# Autodesk Inventor assembly: BobbinGuide
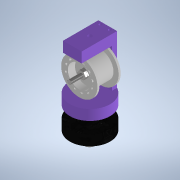
[picture p0: Inventor's stored thumbnail of the model, 180x180]
Saved by Autodesk Inventor 2020.2 (Build 242310000, 310)
## iProperties
Created: 2020-03-09
Part Number: BobbinGuide
Document SubType Name: Assembly
Designer: elmar
Author: elmar
## Documents named in this file (10)
- C:\Users\elmar\OneDrive\Inventor\FourWireBraidingMachine\Carriage.iam
- C:\Users\elmar\OneDrive\Inventor\FourWireBraidingMachine\CarriagePlate.ipt
- C:\Users\elmar\OneDrive\Inventor\FourWireBraidingMachine\SpoolHolder.ipt
- C:\Users\elmar\OneDrive\Inventor\FourWireBraidingMachine\Spool.ipt
- C:\Users\elmar\OneDrive\Inventor\FourWireBraidingMachine\Spring.ipt
- C:\Users\elmar\OneDrive\Documents\Inventor\Content Center Files\R2020\en-US\BS EN 24035\ISO 4035 - M3BS EN.ipt
- C:\Users\elmar\OneDrive\Documents\Inventor\Content Center Files\R2020\en-US\U 2494(1)\Unbrako - M3 x  30(6).ipt
- C:\Users\elmar\OneDrive\Inventor\FourWireBraidingMachine\CarriageGuide.ipt
- C:\Users\elmar\OneDrive\Inventor\FourWireBraidingMachine\SpoolSpringBushing.ipt
- C:\Users\elmar\OneDrive\Inventor\FourWireBraidingMachine\M8_34mmRod.ipt
## Components (10 placed, 9 different names)
1. CarriagePlate:1 — Insert:17
2. CarriageGuide:1
3. SpoolHolder:1 — Insert:14, Insert:15, Insert:16, Insert:17
4. Spool:1 — Mate:1, Mate:5, Insert:15
5. Spring:1 — Mate:1, Mate:5, Mate:6
6. SpoolSpringBushing:1 — Mate:6, Mate:7, Insert:13
7. BS EN 24035 - Metric M3:1 — Insert:9
8. BS EN 24035 - Metric M3:2 — Insert:9, Insert:13
9. Unbrako Hex Socket Cap - Metric M3 x 30:1 — Mate:7, Insert:14
10. M8_34mmRod:1 — Insert:16
## Relationships (10: Insert 6, Mate 4)
- Mate:1: Spool:1 ↔ Spring:1
- Insert:9: BS EN 24035 - Metric M3:1 ↔ BS EN 24035 - Metric M3:2
- Mate:5: Spool:1 ↔ Spring:1
- Mate:6: Spring:1 ↔ SpoolSpringBushing:1
- Mate:7: SpoolSpringBushing:1 ↔ Unbrako Hex Socket Cap - Metric M3 x 30:1
- Insert:13: SpoolSpringBushing:1 ↔ BS EN 24035 - Metric M3:2
- Insert:14: SpoolHolder:1 ↔ Unbrako Hex Socket Cap - Metric M3 x 30:1
- Insert:15: SpoolHolder:1 ↔ Spool:1
- Insert:16: SpoolHolder:1 ↔ M8_34mmRod:1
- Insert:17 (9 mm): CarriagePlate:1 ↔ SpoolHolder:1
